# Autodesk Inventor assembly: Motor Fixture
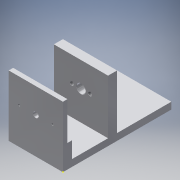
[picture p0: Inventor's stored thumbnail of the model, 180x180]
Saved by Autodesk Inventor 2016 (Build 200138000, 138)
## iProperties
Created: 2015-04-16
Part Number: Motor Fixture
Document SubType Name: Assembly
Designer: jonathan
Mass: 228.301 g
Surface Area: 593.006 cm^2
Volume: 228.301 cm^3
Density: 1 g/cm^3
Author: jonathan
## Documents named in this file (4)
- C:\Users\jonathan\Desktop\Motor\Motor Fixture.iam
- C:\Users\jonathan\Desktop\Motor\Fixture Base.ipt
- C:\Users\jonathan\Desktop\Motor\Fixture Front.ipt
- C:\Users\jonathan\Desktop\Motor\Fixture Center.ipt
## Components (3 placed, 3 different names)
1. Fixture Base:1 — Rigid:1, Cylindrical:1, Cylindrical:2, Mate:1
2. Fixture Front:1 — Rigid:1
3. Fixture Center:1 — Cylindrical:1, Cylindrical:2, Mate:1
## Relationships (4: CylindricalJoint 2, WeldJoint 1, Mate 1)
- Rigid:1 [WeldJoint]: Fixture Base:1 ↔ Fixture Front:1
- Cylindrical:1: Fixture Base:1 ↔ Fixture Center:1
- Cylindrical:2: Fixture Base:1 ↔ Fixture Center:1
- Mate:1: Fixture Base:1 ↔ Fixture Center:1
